# Autodesk Inventor assembly: Morty-01
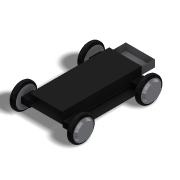
[picture p0: Inventor's stored thumbnail of the model, 180x180]
Saved by Autodesk Inventor 2018 (Build 220112000, 112)
## iProperties
Created: 2017-07-31
Part Number: Morty-01
Document SubType Name: Assembly
Designer: feesmrt
Author: feesmrt
## Documents named in this file (8)
- C:\Users\feesmrt\Documents\NRBDL\Inventor-NRBDL\Morty-01.iam
- C:\Users\feesmrt\Documents\NRBDL\Inventor-NRBDL\20-CASE\20-001-CASE.ipt
- C:\Users\feesmrt\Documents\NRBDL\Inventor-NRBDL\10-SUSP\10-SUSP-03.iam
- C:\Users\feesmrt\Documents\NRBDL\Inventor-NRBDL\10-SUSP\10-SUSP-04_MIR_MIR.iam
- C:\Users\feesmrt\Documents\NRBDL\Inventor-NRBDL\10-SUSP\10-SUSP-03_MIR.iam
- C:\Users\feesmrt\Documents\NRBDL\Inventor-NRBDL\10-SUSP\10-SUSP-04_MIR_MIR_MIR.iam
- C:\Users\feesmrt\Documents\NRBDL\Inventor-NRBDL\20-CASE\20-002-CASE.ipt
- C:\Users\feesmrt\Documents\NRBDL\Inventor-NRBDL\20-CASE\20-003-CASE.ipt
## Components (7 placed, 7 different names)
1. 20-001-CASE:1 — Mate:1, Flush:1, Mate:2, Mate:3, Flush:2, Mate:4, Mate:5, Flush:3, Mate:6, Mate:7, Flush:4, Mate:8, Mate:9, Flush:5, Flush:6, Mate:11
2. 10-SUSP-03:1 [sub-assembly] — Mate:1, Flush:1, Mate:2
3. 10-SUSP-04_MIR_MIR:1 [sub-assembly] — Mate:3, Flush:2, Mate:4
4. 10-SUSP-03_MIR:1 [sub-assembly] — Mate:7, Flush:4, Mate:8
5. 10-SUSP-04_MIR_MIR_MIR:1 [sub-assembly] — Mate:5, Flush:3, Mate:6
6. 20-002-CASE:1 — Mate:9, Flush:5, Flush:6
7. 20-003-CASE:1 — Mate:10, Mate:11
## Relationships (17: Mate 11, Flush 6)
- Mate:1: 20-001-CASE:1 ↔ 10-SUSP-03:1
- Flush:1: 20-001-CASE:1 ↔ 10-SUSP-03:1
- Mate:2: 20-001-CASE:1 ↔ 10-SUSP-03:1
- Mate:3: 20-001-CASE:1 ↔ 10-SUSP-04_MIR_MIR:1
- Flush:2: 20-001-CASE:1 ↔ 10-SUSP-04_MIR_MIR:1
- Mate:4: 20-001-CASE:1 ↔ 10-SUSP-04_MIR_MIR:1
- Mate:5: 20-001-CASE:1 ↔ 10-SUSP-04_MIR_MIR_MIR:1
- Flush:3: 20-001-CASE:1 ↔ 10-SUSP-04_MIR_MIR_MIR:1
- Mate:6: 20-001-CASE:1 ↔ 10-SUSP-04_MIR_MIR_MIR:1
- Mate:7: 20-001-CASE:1 ↔ 10-SUSP-03_MIR:1
- Flush:4: 20-001-CASE:1 ↔ 10-SUSP-03_MIR:1
- Mate:8: 20-001-CASE:1 ↔ 10-SUSP-03_MIR:1
- Mate:9: 20-001-CASE:1 ↔ 20-002-CASE:1
- Flush:5: 20-001-CASE:1 ↔ 20-002-CASE:1
- Flush:6: 20-001-CASE:1 ↔ 20-002-CASE:1
- Mate:10: 20-003-CASE:1
- Mate:11 (10 mm): 20-001-CASE:1 ↔ 20-003-CASE:1
